# Autodesk Inventor assembly: 10-06-01 ansamblu display
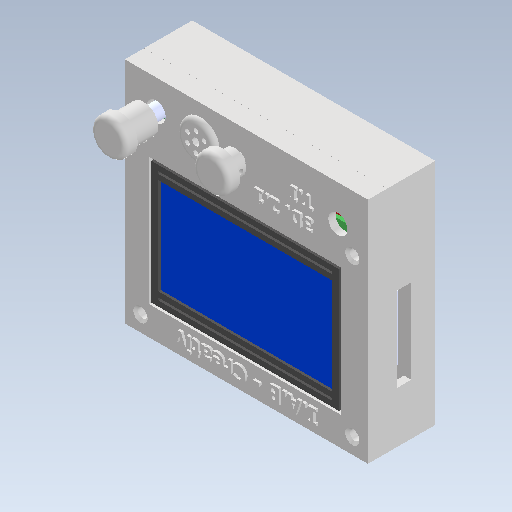
[picture p0: Inventor's stored thumbnail of the model, 512x512]
Saved by Autodesk Inventor 2020 (Build 240168000, 168)
## iProperties
Created: 2019-11-09
Part Number: 10-06-01 ansamblu display
Document SubType Name: Assembly
Designer: iuliu
Author: iuliu
## Documents named in this file (7)
- Z:\I.A.B\Proiecte\0008 I.A.B 3D 2.1 Imprimanta aracet Metal\10 Mecanic\0008-10-11 ansamblu display.iam
- Z:\I.A.B\Proiecte\0008 I.A.B 3D 2.1 Imprimanta aracet Metal\20 Electric\0008-20-1011 ReprapDiscountFullGraphicSmartController-Robotale_Dummy.ipt
- Z:\I.A.B\Proiecte\0008 I.A.B 3D 2.1 Imprimanta aracet Metal\10 Mecanic\0008-10-039 carcasa spate.ipt
- Z:\I.A.B\Proiecte\0008 I.A.B 3D 2.1 Imprimanta aracet Metal\10 Mecanic\0008-10-038  carcasa Fata.ipt
- Z:\I.A.B\Proiecte\0008 I.A.B 3D 2.1 Imprimanta aracet Metal\10 Mecanic\0008-10-040 Buotn_Urgenta.ipt
- Z:\I.A.B\Proiecte\0008 I.A.B 3D 2.1 Imprimanta aracet Metal\10 Mecanic\0008-10-041 Ciuperca.ipt
- Z:\I.A.B\Proiecte\0008 I.A.B 3D 2.1 Imprimanta aracet Metal\10 Mecanic\0008-10-042 Joistic.ipt
## Components (6 placed, 6 different names)
1. 10-06-03 ReprapDiscountFullGraphicSmartController-Robotale_Dummy.ipt:1 — Flush:1, Flush:2, Flush:3, Mate:1, Mate:2, Insert:3
2. 0008-10-039 carcasa spate.ipt:2 — Flush:1, Flush:2, Flush:3, Mate:3, Angle:1
3. 0008-10-038  carcasa Fata.ipt:3 — Mate:1, Mate:2, Mate:3, Insert:1
4. 0008-10-040 Buotn_Urgenta.ipt:4 — Insert:1, Insert:2
5. 0008-10-041 Ciuperca.ipt:5 — Insert:2
6. 0008-10-042 Joistic.ipt:6 — Insert:3
## Relationships (10: Flush 3, Mate 3, Insert 3, Angle 1)
- Flush:1: 10-06-03 ReprapDiscountFullGraphicSmartController-Robotale_Dummy.ipt:1 ↔ 0008-10-039 carcasa spate.ipt:2
- Flush:2 (4 mm): 10-06-03 ReprapDiscountFullGraphicSmartController-Robotale_Dummy.ipt:1 ↔ 0008-10-039 carcasa spate.ipt:2
- Flush:3 (4 mm): 10-06-03 ReprapDiscountFullGraphicSmartController-Robotale_Dummy.ipt:1 ↔ 0008-10-039 carcasa spate.ipt:2
- Mate:1: 10-06-03 ReprapDiscountFullGraphicSmartController-Robotale_Dummy.ipt:1 ↔ 0008-10-038  carcasa Fata.ipt:3
- Mate:2: 10-06-03 ReprapDiscountFullGraphicSmartController-Robotale_Dummy.ipt:1 ↔ 0008-10-038  carcasa Fata.ipt:3
- Mate:3: 0008-10-039 carcasa spate.ipt:2 ↔ 0008-10-038  carcasa Fata.ipt:3
- Insert:1: 0008-10-038  carcasa Fata.ipt:3 ↔ 0008-10-040 Buotn_Urgenta.ipt:4
- Insert:2: 0008-10-040 Buotn_Urgenta.ipt:4 ↔ 0008-10-041 Ciuperca.ipt:5
- Insert:3: 10-06-03 ReprapDiscountFullGraphicSmartController-Robotale_Dummy.ipt:1 ↔ 0008-10-042 Joistic.ipt:6
- Angle:1 (0 deg): 0008-10-039 carcasa spate.ipt:2
